# Autodesk Inventor assembly: 000.005 - Блок АКБ
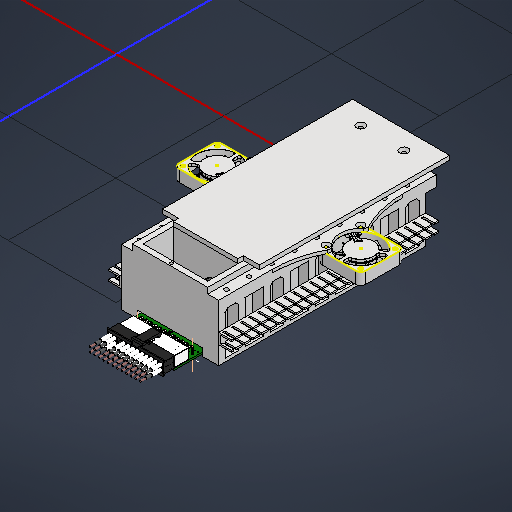
[picture p0: Inventor's stored thumbnail of the model, 512x512]
Saved by Autodesk Inventor 2025 (Build 290162000, 162)
## iProperties
Created: 2024-08-02
Part Number: 000.005 - Блок АКБ
Document SubType Name: Assembly
Designer: IvanPetrov
Author: IvanPetrov
## Documents named in this file (9)
- D:\Projects\OmniBot\design\000.005 - Блок АКБ.iam
- D:\Projects\OmniBot\design\000.005.001 - Корпус.ipt
- D:\Projects\OmniBot\design\standart_components\NUCLEO.ipt
- D:\Projects\OmniBot\design\standart_components\Bosch Relay 12Vdc - 30A SPST.ipt
- D:\Projects\OmniBot\design\000.005.002 - Кабель канал.ipt
- D:\Projects\OmniBot\design\000.007 - Монитор заряда АКБ.iam
- D:\Projects\OmniBot\design\standart_components\atx\ATX-Main-23-Pin\ATX-Main-23-Pin.iam
- D:\Projects\OmniBot\design\standart_components\fan\fan4040\fan4040.iam
- D:\Projects\OmniBot\design\000.005.003 - Крышка.ipt
## Components (11 placed, 8 different names)
1. 000.005.001 - Корпус:1 — Касательность:2, Угол:2, Совмещение:3, Совмещение:4, Совмещение:5, Совмещение:6, Совмещение:10, Совмещение:12, Заподлицо:6, Совмещение:13, Заподлицо:8, Совмещение:15, Совмещение:16, Совмещение:18, Совмещение:19, Совмещение:20, Совмещение:21, Совмещение:22, Совмещение:23, Совмещение:24, Совмещение:25, Заподлицо:11, Совмещение:26
2. NUCLEO:1 — Касательность:2, Угол:2, Заподлицо:1, Совмещение:1, Совмещение:2, Совмещение:3, Совмещение:10
3. NUCLEO:2 — Заподлицо:1, Совмещение:1, Совмещение:2
4. Bosch Relay 12Vdc - 30A SPST:1 — Совмещение:4, Совмещение:5, Совмещение:6
5. 000.005.002 - Кабель канал:1 — Совмещение:12, Заподлицо:6, Заподлицо:7
6. 000.005.002 - Кабель канал:2 — Совмещение:13, Заподлицо:7, Заподлицо:8
7. 000.007 - Монитор заряда АКБ:1 [sub-assembly] — Совмещение:15, Совмещение:16, Заподлицо:9, Заподлицо:10, Совмещение:17, Совмещение:26
8. ATX-Main-23-Pin:1 [sub-assembly] — Заподлицо:9, Заподлицо:10, Совмещение:17
9. fan4040:1 [sub-assembly] — Совмещение:21, Совмещение:22, Совмещение:23
10. fan4040:2 [sub-assembly] — Совмещение:18, Совмещение:19, Совмещение:20
11. 000.005.003 - Крышка:1 — Совмещение:24, Совмещение:25, Заподлицо:11
## Relationships (30: Mate 21, Flush 7, Tangent 1, Angle 1)
- Касательность:2 [Tangent]: 000.005.001 - Корпус:1 ↔ NUCLEO:1
- Угол:2 [Angle] (0 deg): 000.005.001 - Корпус:1 ↔ NUCLEO:1
- Заподлицо:1 [Flush]: NUCLEO:1 ↔ NUCLEO:2
- Совмещение:1 [Mate] (20 mm): NUCLEO:1 ↔ NUCLEO:2
- Совмещение:2 [Mate]: NUCLEO:1 ↔ NUCLEO:2
- Совмещение:3 [Mate]: 000.005.001 - Корпус:1 ↔ NUCLEO:1
- Совмещение:4 [Mate]: 000.005.001 - Корпус:1 ↔ Bosch Relay 12Vdc - 30A SPST:1
- Совмещение:5 [Mate]: 000.005.001 - Корпус:1 ↔ Bosch Relay 12Vdc - 30A SPST:1
- Совмещение:6 [Mate]: 000.005.001 - Корпус:1 ↔ Bosch Relay 12Vdc - 30A SPST:1
- Совмещение:10 [Mate] (1 mm): 000.005.001 - Корпус:1 ↔ NUCLEO:1
- Совмещение:12 [Mate]: 000.005.001 - Корпус:1 ↔ 000.005.002 - Кабель канал:1
- Заподлицо:6 [Flush]: 000.005.001 - Корпус:1 ↔ 000.005.002 - Кабель канал:1
- Совмещение:13 [Mate]: 000.005.001 - Корпус:1 ↔ 000.005.002 - Кабель канал:2
- Заподлицо:7 [Flush]: 000.005.002 - Кабель канал:1 ↔ 000.005.002 - Кабель канал:2
- Заподлицо:8 [Flush]: 000.005.001 - Корпус:1 ↔ 000.005.002 - Кабель канал:2
- Совмещение:15 [Mate]: 000.005.001 - Корпус:1 ↔ 000.007 - Монитор заряда АКБ:1
- Совмещение:16 [Mate]: 000.005.001 - Корпус:1 ↔ 000.007 - Монитор заряда АКБ:1
- Заподлицо:9 [Flush]: 000.007 - Монитор заряда АКБ:1 ↔ ATX-Main-23-Pin:1
- Заподлицо:10 [Flush]: 000.007 - Монитор заряда АКБ:1 ↔ ATX-Main-23-Pin:1
- Совмещение:17 [Mate]: 000.007 - Монитор заряда АКБ:1 ↔ ATX-Main-23-Pin:1
- Совмещение:18 [Mate]: 000.005.001 - Корпус:1 ↔ fan4040:2
- Совмещение:19 [Mate]: 000.005.001 - Корпус:1 ↔ fan4040:2
- Совмещение:20 [Mate]: 000.005.001 - Корпус:1 ↔ fan4040:2
- Совмещение:21 [Mate]: 000.005.001 - Корпус:1 ↔ fan4040:1
- Совмещение:22 [Mate]: 000.005.001 - Корпус:1 ↔ fan4040:1
- Совмещение:23 [Mate]: 000.005.001 - Корпус:1 ↔ fan4040:1
- Совмещение:24 [Mate]: 000.005.001 - Корпус:1 ↔ 000.005.003 - Крышка:1
- Совмещение:25 [Mate]: 000.005.001 - Корпус:1 ↔ 000.005.003 - Крышка:1
- Заподлицо:11 [Flush]: 000.005.001 - Корпус:1 ↔ 000.005.003 - Крышка:1
- Совмещение:26 [Mate] (-2 mm): 000.005.001 - Корпус:1 ↔ 000.007 - Монитор заряда АКБ:1
